# Autodesk Inventor assembly: BGgerüst_2_trajan20_21
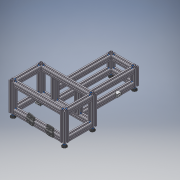
[picture p0: Inventor's stored thumbnail of the model, 180x180]
Saved by Autodesk Inventor 2022.2 (Build 262287000, 287)
## iProperties
Company: HTBLA Kaindorf
RuleStatus: InUse
Created: 2022-08-20
Part Number: BGgerüst_2_trajan20_21
Project: Zeichenmaschine_v2
Material: Generisch
Description: 102
Document SubType Name: Assembly
Designer: trajan20
AfterDocNew0: iProperties-Editor_aufrufen
Author: jan
Keywords: 2021
## Documents named in this file (5)
- C:\Users\jan\Documents\DrawMachine\DrawMachineConstruction\Projekt\Zeichenmaschine_v2\BG102_gerüst_2_trajan20_21_Zeichenmaschine_v2.iam
- C:\Users\jan\Documents\DrawMachine\DrawMachineConstruction\Projekt\Zeichenmaschine_v2\step dateien\gerüst_item_2022-07-24_alu_construct_Projekt_ID-a403a0fdf3734c62922616c2a250de6220_1.ipt
- C:\Users\jan\Documents\DrawMachine\DrawMachineConstruction\Projekt\Zeichenmaschine_v2\step dateien\Magnetschnäpper _093094.ipt
- C:\Users\jan\Documents\DrawMachine\DrawMachineConstruction\Projekt\Zeichenmaschine_v2\step dateien\scharnier_095K2020L00.ipt
- C:\Users\jan\Documents\DrawMachine\DrawMachineConstruction\Projekt\Zeichenmaschine_v2\step dateien\uniblock_094411m4.ipt
## Components (5 placed, 4 different names)
1. gerüst_item_2022-07-24_alu_construct_Projekt_ID-a403a0fdf3734c62922616c2a250de6220_1:1 — Passend:1, Passend:2, Passend:3, Passend:4, Passend:5, Passend:6
2. Magnetschnäpper _093094:1 — Passend:1
3. scharnier_095K2020L00:1 — Passend:2, Passend:6
4. scharnier_095K2020L00:2 — Passend:3, Passend:4, Passend:5
5. uniblock_094411m4:1
## Relationships (6: Mate 6)
- Passend:1 [Mate]: gerüst_item_2022-07-24_alu_construct_Projekt_ID-a403a0fdf3734c62922616c2a250de6220_1:1 ↔ Magnetschnäpper _093094:1
- Passend:2 [Mate]: gerüst_item_2022-07-24_alu_construct_Projekt_ID-a403a0fdf3734c62922616c2a250de6220_1:1 ↔ scharnier_095K2020L00:1
- Passend:3 [Mate]: gerüst_item_2022-07-24_alu_construct_Projekt_ID-a403a0fdf3734c62922616c2a250de6220_1:1 ↔ scharnier_095K2020L00:2
- Passend:4 [Mate] (2.5 mm): gerüst_item_2022-07-24_alu_construct_Projekt_ID-a403a0fdf3734c62922616c2a250de6220_1:1 ↔ scharnier_095K2020L00:2
- Passend:5 [Mate] (2.5 mm): gerüst_item_2022-07-24_alu_construct_Projekt_ID-a403a0fdf3734c62922616c2a250de6220_1:1 ↔ scharnier_095K2020L00:2
- Passend:6 [Mate] (2.5 mm): gerüst_item_2022-07-24_alu_construct_Projekt_ID-a403a0fdf3734c62922616c2a250de6220_1:1 ↔ scharnier_095K2020L00:1
